# Autodesk Inventor assembly: RollerAssembely
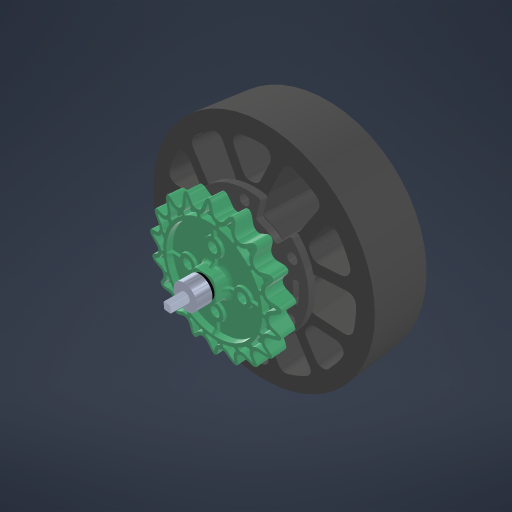
[picture p0: Inventor's stored thumbnail of the model, 512x512]
Saved by Autodesk Inventor 2023 (Build 270158000, 158)
## iProperties
Created: 2022-11-12
Part Number: RollerAssembely
Document SubType Name: Assembly
Designer: alex
Author: alex
## Documents named in this file (6)
- C:\Users\alex\Documents\GitHub\4067X_spin_up_cad\RollerAssembely.iam
- C:\Users\alex\Documents\GitHub\4067X_spin_up_cad\WithAdapter4Inch60A.iam
- C:\Users\alex\Documents\GitHub\4067X_spin_up_cad\Library\Motion\Sprockets\HS 18T Sprocket, Square.ipt
- C:\Users\alex\Documents\GitHub\4067X_spin_up_cad\Library\Motion\Shaft LS\Shaft LS 3.0 in.ipt
- C:\Users\alex\Documents\GitHub\4067X_spin_up_cad\Library\Motion\Shaft LS.ipt
- C:\Users\alex\Documents\GitHub\4067X_spin_up_cad\Library\Motion\Shaft Collar with Set Screw.ipt
## Components (4 placed, 4 different names)
1. WithAdapter4Inch60A:1 [sub-assembly] — Insert:1, Rotation:1
2. HS 18T Sprocket, Square:1 — Insert:1, Rotation:1, Mate:1, Mate:2, Insert:2
3. Shaft LS 3.0 in:1 — Mate:1, Mate:2
4. Shaft Collar with Set Screw:1 — Insert:2
## Relationships (5: Insert 2, Mate 2, RelateRotation 1)
- Insert:1: WithAdapter4Inch60A:1 ↔ HS 18T Sprocket, Square:1
- Rotation:1 [RelateRotation] (1 ul): WithAdapter4Inch60A:1 ↔ HS 18T Sprocket, Square:1
- Mate:1: HS 18T Sprocket, Square:1 ↔ Shaft LS 3.0 in:1
- Mate:2: HS 18T Sprocket, Square:1 ↔ Shaft LS 3.0 in:1
- Insert:2: HS 18T Sprocket, Square:1 ↔ Shaft Collar with Set Screw:1
